# Autodesk Inventor assembly: 로드셀 케이스 조립
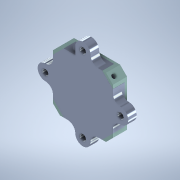
[picture p0: Inventor's stored thumbnail of the model, 180x180]
Saved by Autodesk Inventor 2021 (Build 250183000, 183)
## iProperties
Created: 2021-08-10
Part Number: 로드셀 케이스 조립
Document SubType Name: Assembly
Designer: Dongyoon
Author: Dongyoon
## Documents named in this file (3)
- C:\Users\Dongyoon\Desktop\인벤터 모델링\로드셀 케이스 조립.iam
- C:\Users\Dongyoon\Desktop\인벤터 모델링\로드셀 케이스2.ipt
- C:\Users\Dongyoon\Desktop\인벤터 모델링\로드셀 케이스2-1.ipt
## Components (2 placed, 2 different names)
1. 로드셀 케이스2:1 — 메이트:1, 메이트:2, 메이트:3
2. 로드셀 케이스2-1:1 — 메이트:1, 메이트:2, 메이트:3
## Relationships (3: Mate 3)
- 메이트:1 [Mate]: 로드셀 케이스2:1 ↔ 로드셀 케이스2-1:1
- 메이트:2 [Mate]: 로드셀 케이스2:1 ↔ 로드셀 케이스2-1:1
- 메이트:3 [Mate]: 로드셀 케이스2:1 ↔ 로드셀 케이스2-1:1
